# Autodesk Inventor assembly: Assembly1
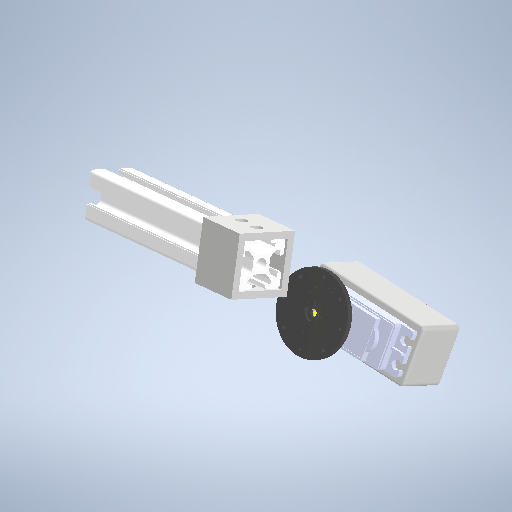
[picture p0: Inventor's stored thumbnail of the model, 512x512]
Saved by Autodesk Inventor 2025 (Build 290162000, 162)
## iProperties
Created: 2024-05-25
Part Number: Assembly1
Document SubType Name: Assembly
Designer: hifzh
Author: hifzh
## Documents named in this file (7)
- C:\Users\hifzh\final_year\Design\TA-Design\Assembly1.iam
- C:\Users\hifzh\final_year\Design\TA-Design\Aluminium2020-connector.ipt
- C:\Users\hifzh\final_year\Design\TA-Design\servo_to_links1.ipt
- C:\Users\hifzh\final_year\Design\TA-Design\servo_to_links2.ipt
- C:\Users\hifzh\final_year\Design\TA-Design\servos.ipt
- C:\Users\hifzh\final_year\Design\TA-Design\20X20 - Aluminium Profile v1.ipt
- C:\Users\hifzh\final_year\Design\TA-Design\futaba_horn_35mm_round v1.ipt
## Components (6 placed, 6 different names)
1. Aluminium2020-connector:1 — Mate:4, Mate:5
2. servo_to_links1:1 — Mate:1, Mate:2, Mate:3
3. servo_to_links2:1
4. servos:1 — Mate:1, Mate:2, Mate:3, Insert:1
5. 20X20 - Aluminium Profile v1:1 — Mate:4, Mate:5
6. futaba_horn_35mm_round v1:1 — Insert:1
## Relationships (6: Mate 5, Insert 1)
- Mate:1: servo_to_links1:1 ↔ servos:1
- Mate:2: servo_to_links1:1 ↔ servos:1
- Mate:3: servo_to_links1:1 ↔ servos:1
- Mate:4: Aluminium2020-connector:1 ↔ 20X20 - Aluminium Profile v1:1
- Mate:5: Aluminium2020-connector:1 ↔ 20X20 - Aluminium Profile v1:1
- Insert:1: servos:1 ↔ futaba_horn_35mm_round v1:1
